# Autodesk Inventor assembly: maket02
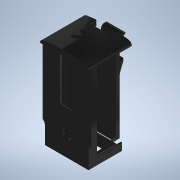
[picture p0: Inventor's stored thumbnail of the model, 180x180]
Saved by Autodesk Inventor 2020 (Build 240168000, 168)
## iProperties
Created: 2024-02-27
Part Number: maket02
Document SubType Name: Assembly
Designer: 4s
Author: 4s
## Documents named in this file (3)
- C:\Users\4s\Documents\Inventor models\Asterisk\robot_v2\Bat_mount\maket02.iam
- C:\Users\4s\Documents\Inventor models\Asterisk\robot_v2\Bat_mount\bat_mount003.ipt
- C:\Users\4s\Documents\Inventor models\Asterisk\robot_v2\Bat_mount\bat_lock03_straight.ipt
## Components (2 placed, 2 different names)
1. bat_mount003:1 — Совмещение:1, Угол:1, Заподлицо:1
2. bat_lock03_straight:1 — Совмещение:1, Угол:1, Заподлицо:1
## Relationships (3: Mate 1, Angle 1, Flush 1)
- Совмещение:1 [Mate] (1 mm): bat_mount003:1 ↔ bat_lock03_straight:1
- Угол:1 [Angle] (0 deg): bat_mount003:1 ↔ bat_lock03_straight:1
- Заподлицо:1 [Flush]: bat_mount003:1 ↔ bat_lock03_straight:1
